# Autodesk Inventor assembly: rope winding mechanism
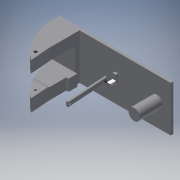
[picture p0: Inventor's stored thumbnail of the model, 180x180]
Saved by Autodesk Inventor 2019 (Build 230136000, 136)
## iProperties
Created: 2020-02-27
Part Number: rope winding mechanism
Document SubType Name: Assembly
Designer: Rajesh
Author: Rajesh
## Documents named in this file (4)
- C:\Users\Rajesh\Desktop\New folder\rope winding mechanism.iam
- C:\Users\Rajesh\Desktop\New folder\servo part.ipt
- C:\Users\Rajesh\Desktop\New folder\rope holder.ipt
- C:\Users\Rajesh\Desktop\New folder\base part.ipt
## Components (3 placed, 3 different names)
1. servo part:1 — Mate:1, Mate:2, Mate:3, Mate:4, Mate:5
2. rope holder:1 — Mate:1, Mate:2
3. base part:1 — Mate:3, Mate:4, Mate:5
## Relationships (5: Mate 5)
- Mate:1: servo part:1 ↔ rope holder:1
- Mate:2: servo part:1 ↔ rope holder:1
- Mate:3: servo part:1 ↔ base part:1
- Mate:4: servo part:1 ↔ base part:1
- Mate:5: servo part:1 ↔ base part:1
